# Autodesk Inventor assembly: Final Projectile Launcher
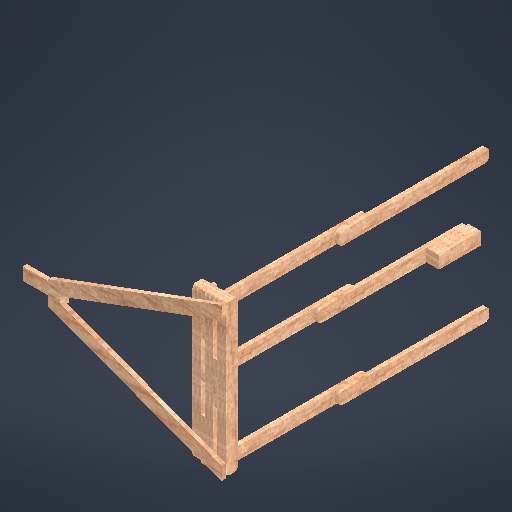
[picture p0: Inventor's stored thumbnail of the model, 512x512]
Saved by Autodesk Inventor 2026 (Build 300175000, 175)
## iProperties
Created: 2023-09-26
Part Number: Final Projectile Launcher
Document SubType Name: Assembly
Designer: Nick
Author: Nick
## Documents named in this file (4)
- C:\Users\Nick\Documents\Inventor\Inventor\MMAE 100 Project\Final Projectile Launcher.iam
- C:\Users\Nick\Documents\Inventor\Inventor\MMAE 100 Project\Projectile Launcher Popsicle Stick.ipt
- C:\Users\Nick\Documents\Inventor\Inventor\MMAE 100 Project\Projectile Launcher Partial Popsicle Stick.ipt
- C:\Users\Nick\Documents\Inventor\Inventor\MMAE 100 Project\Projectile Launcher Back.ipt
## Components (20 placed, 3 different names)
1. Projectile Launcher Popsicle Stick:1 — Mate:1, Flush:1, Flush:2, Mate:2, Flush:3, Flush:4, Mate:3, Flush:5, Flush:6, Mate:4, Flush:7
2. Projectile Launcher Popsicle Stick:2 — Mate:1, Flush:1, Flush:2
3. Projectile Launcher Popsicle Stick:3 — Mate:6, Flush:11, Flush:12, Mate:7, Flush:13, Flush:26, Flush:27
4. Projectile Launcher Popsicle Stick:4 — Mate:5, Flush:9, Flush:10, Mate:18, Flush:32, Flush:33, Flush:35
5. Projectile Launcher Popsicle Stick:5 — Mate:7, Flush:13, Flush:14, Mate:8, Mate:9, Flush:15, Flush:16, Mate:11, Flush:19, Flush:20, Mate:14, Flush:23
6. Projectile Launcher Popsicle Stick:6 — Mate:4, Flush:7, Flush:8, Mate:5, Flush:9, Flush:10
7. Projectile Launcher Popsicle Stick:7 — Mate:10, Flush:17, Flush:18
8. Projectile Launcher Popsicle Stick:8 — Mate:8, Mate:9, Flush:15, Flush:16, Mate:10, Flush:17, Flush:18
9. Projectile Launcher Popsicle Stick:9 — Mate:11, Flush:19, Flush:20, Mate:12, Flush:21, Flush:22
10. Projectile Launcher Popsicle Stick:10 — Mate:12, Flush:21, Flush:22
11. Projectile Launcher Popsicle Stick:14 — Mate:15, Flush:25, Flush:26, Mate:16, Flush:28
12. Projectile Launcher Popsicle Stick:16 — Mate:16, Flush:27, Flush:28, Flush:29, Flush:31
13. Projectile Launcher Partial Popsicle Stick:1 — Mate:3, Flush:5, Flush:6, Mate:13
14. Projectile Launcher Partial Popsicle Stick:2 — Mate:17, Flush:30, Flush:31
15. Projectile Launcher Partial Popsicle Stick:3 — Mate:19, Flush:34, Flush:35, Mate:20, Flush:36, Flush:37
16. Projectile Launcher Partial Popsicle Stick:4 — Mate:14, Flush:23, Flush:24, Mate:15, Flush:25
17. Projectile Launcher Partial Popsicle Stick:6 — Mate:2, Flush:3, Flush:4, Flush:8, Mate:6, Flush:11, Flush:12, Flush:14, Flush:24
18. Projectile Launcher Partial Popsicle Stick:7 — Mate:18, Flush:32, Flush:33, Mate:19, Flush:34
19. Projectile Launcher Partial Popsicle Stick:8 — Mate:20, Flush:36, Flush:37
20. Projectile Launcher Back:1 — Mate:13, Flush:29, Mate:17, Flush:30
## Relationships (57: Flush 37, Mate 20)
- Mate:1: Projectile Launcher Popsicle Stick:1 ↔ Projectile Launcher Popsicle Stick:2
- Flush:1: Projectile Launcher Popsicle Stick:1 ↔ Projectile Launcher Popsicle Stick:2
- Flush:2: Projectile Launcher Popsicle Stick:1 ↔ Projectile Launcher Popsicle Stick:2
- Mate:2: Projectile Launcher Popsicle Stick:1 ↔ Projectile Launcher Partial Popsicle Stick:6
- Flush:3: Projectile Launcher Popsicle Stick:1 ↔ Projectile Launcher Partial Popsicle Stick:6
- Flush:4: Projectile Launcher Popsicle Stick:1 ↔ Projectile Launcher Partial Popsicle Stick:6
- Mate:3: Projectile Launcher Popsicle Stick:1 ↔ Projectile Launcher Partial Popsicle Stick:1
- Flush:5: Projectile Launcher Popsicle Stick:1 ↔ Projectile Launcher Partial Popsicle Stick:1
- Flush:6: Projectile Launcher Popsicle Stick:1 ↔ Projectile Launcher Partial Popsicle Stick:1
- Mate:4: Projectile Launcher Popsicle Stick:1 ↔ Projectile Launcher Popsicle Stick:6
- Flush:7: Projectile Launcher Popsicle Stick:1 ↔ Projectile Launcher Popsicle Stick:6
- Flush:8 (52.3875 mm): Projectile Launcher Popsicle Stick:6 ↔ Projectile Launcher Partial Popsicle Stick:6
- Mate:5: Projectile Launcher Popsicle Stick:4 ↔ Projectile Launcher Popsicle Stick:6
- Flush:9: Projectile Launcher Popsicle Stick:4 ↔ Projectile Launcher Popsicle Stick:6
- Flush:10 (82.55 mm): Projectile Launcher Popsicle Stick:4 ↔ Projectile Launcher Popsicle Stick:6
- Mate:6: Projectile Launcher Popsicle Stick:3 ↔ Projectile Launcher Partial Popsicle Stick:6
- Flush:11: Projectile Launcher Popsicle Stick:3 ↔ Projectile Launcher Partial Popsicle Stick:6
- Flush:12: Projectile Launcher Popsicle Stick:3 ↔ Projectile Launcher Partial Popsicle Stick:6
- Mate:7: Projectile Launcher Popsicle Stick:3 ↔ Projectile Launcher Popsicle Stick:5
- Flush:13: Projectile Launcher Popsicle Stick:3 ↔ Projectile Launcher Popsicle Stick:5
- Flush:14: Projectile Launcher Popsicle Stick:5 ↔ Projectile Launcher Partial Popsicle Stick:6
- Mate:8: Projectile Launcher Popsicle Stick:5 ↔ Projectile Launcher Popsicle Stick:8
- Mate:9: Projectile Launcher Popsicle Stick:5 ↔ Projectile Launcher Popsicle Stick:8
- Flush:15: Projectile Launcher Popsicle Stick:5 ↔ Projectile Launcher Popsicle Stick:8
- Flush:16: Projectile Launcher Popsicle Stick:5 ↔ Projectile Launcher Popsicle Stick:8
- Mate:10: Projectile Launcher Popsicle Stick:7 ↔ Projectile Launcher Popsicle Stick:8
- Flush:17: Projectile Launcher Popsicle Stick:7 ↔ Projectile Launcher Popsicle Stick:8
- Flush:18 (88.9 mm): Projectile Launcher Popsicle Stick:7 ↔ Projectile Launcher Popsicle Stick:8
- Mate:11: Projectile Launcher Popsicle Stick:5 ↔ Projectile Launcher Popsicle Stick:9
- Flush:19: Projectile Launcher Popsicle Stick:5 ↔ Projectile Launcher Popsicle Stick:9
- Flush:20: Projectile Launcher Popsicle Stick:5 ↔ Projectile Launcher Popsicle Stick:9
- Mate:12: Projectile Launcher Popsicle Stick:9 ↔ Projectile Launcher Popsicle Stick:10
- Flush:21: Projectile Launcher Popsicle Stick:9 ↔ Projectile Launcher Popsicle Stick:10
- Flush:22 (-88.9 mm): Projectile Launcher Popsicle Stick:9 ↔ Projectile Launcher Popsicle Stick:10
- Mate:13: Projectile Launcher Partial Popsicle Stick:1 ↔ Projectile Launcher Back:1
- Mate:14: Projectile Launcher Popsicle Stick:5 ↔ Projectile Launcher Partial Popsicle Stick:4
- Flush:23: Projectile Launcher Popsicle Stick:5 ↔ Projectile Launcher Partial Popsicle Stick:4
- Flush:24 (42.037 mm): Projectile Launcher Partial Popsicle Stick:4 ↔ Projectile Launcher Partial Popsicle Stick:6
- Mate:15: Projectile Launcher Popsicle Stick:14 ↔ Projectile Launcher Partial Popsicle Stick:4
- Flush:25: Projectile Launcher Popsicle Stick:14 ↔ Projectile Launcher Partial Popsicle Stick:4
- Flush:26: Projectile Launcher Popsicle Stick:3 ↔ Projectile Launcher Popsicle Stick:14
- Mate:16: Projectile Launcher Popsicle Stick:14 ↔ Projectile Launcher Popsicle Stick:16
- Flush:27: Projectile Launcher Popsicle Stick:3 ↔ Projectile Launcher Popsicle Stick:16
- Flush:28: Projectile Launcher Popsicle Stick:14 ↔ Projectile Launcher Popsicle Stick:16
- Flush:29: Projectile Launcher Popsicle Stick:16 ↔ Projectile Launcher Back:1
- Mate:17: Projectile Launcher Partial Popsicle Stick:2 ↔ Projectile Launcher Back:1
- Flush:30: Projectile Launcher Partial Popsicle Stick:2 ↔ Projectile Launcher Back:1
- Flush:31 (52.07 mm): Projectile Launcher Popsicle Stick:16 ↔ Projectile Launcher Partial Popsicle Stick:2
- Mate:18: Projectile Launcher Popsicle Stick:4 ↔ Projectile Launcher Partial Popsicle Stick:7
- Flush:32: Projectile Launcher Popsicle Stick:4 ↔ Projectile Launcher Partial Popsicle Stick:7
- Flush:33: Projectile Launcher Popsicle Stick:4 ↔ Projectile Launcher Partial Popsicle Stick:7
- Mate:19: Projectile Launcher Partial Popsicle Stick:3 ↔ Projectile Launcher Partial Popsicle Stick:7
- Flush:34: Projectile Launcher Partial Popsicle Stick:3 ↔ Projectile Launcher Partial Popsicle Stick:7
- Flush:35: Projectile Launcher Popsicle Stick:4 ↔ Projectile Launcher Partial Popsicle Stick:3
- Mate:20: Projectile Launcher Partial Popsicle Stick:3 ↔ Projectile Launcher Partial Popsicle Stick:8
- Flush:36: Projectile Launcher Partial Popsicle Stick:3 ↔ Projectile Launcher Partial Popsicle Stick:8
- Flush:37: Projectile Launcher Partial Popsicle Stick:3 ↔ Projectile Launcher Partial Popsicle Stick:8
